# Autodesk Inventor assembly: motor_a;;
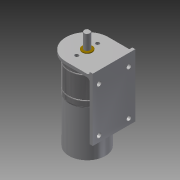
[picture p0: Inventor's stored thumbnail of the model, 180x180]
Saved by Autodesk Inventor 2015 (Build 190159000, 159)
## iProperties
Created: 2015-03-18
Part Number: motor_a;;
Document SubType Name: Assembly
Designer: Marcin
Author: Marcin
## Documents named in this file (3)
- C:\Users\Kuba\Dysk Google\synergia\Synergolf\model\GOLF\motor_all.iam
- C:\Users\Kuba\Dysk Google\synergia\Synergolf\model\GOLF\motor_dc.ipt
- C:\Users\Kuba\Dysk Google\synergia\Synergolf\model\GOLF\console.ipt
## Components (2 placed, 2 different names)
1. motor_dc:1 — Równoległy:1, Równoległy:2, Równoległy:3, Równoległy:4, Równoległy:5
2. console:1 — Równoległy:4, Równoległy:5
## Relationships (5: Flush 5)
- Równoległy:1 [Flush]: motor_dc:1
- Równoległy:2 [Flush]: motor_dc:1
- Równoległy:3 [Flush]: motor_dc:1
- Równoległy:4 [Flush]: motor_dc:1 ↔ console:1
- Równoległy:5 [Flush]: motor_dc:1 ↔ console:1
